# Autodesk Inventor assembly: Solar Array
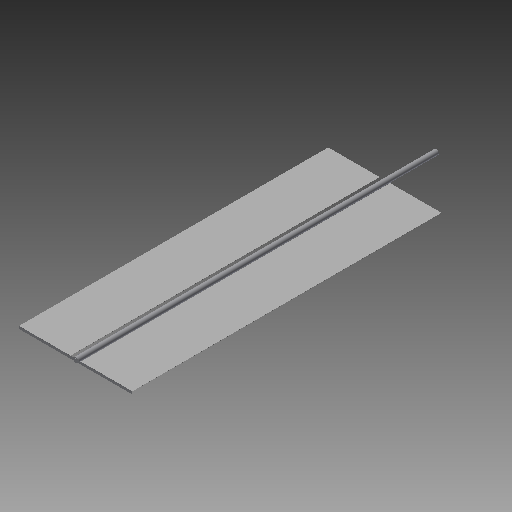
[picture p0: Inventor's stored thumbnail of the model, 512x512]
Saved by Autodesk Inventor 2017.2 (Build 212233000, 233)
## iProperties
Created: 2017-03-31
Part Number: Solar Array
Document SubType Name: Assembly
Designer: haden
Author: haden
## Documents named in this file (3)
- C:\Users\haden\Desktop\Asteroid-Mining-Project\CAD model\Solar Module\Solar Array.iam
- C:\Users\haden\Desktop\Asteroid-Mining-Project\CAD model\Solar Module\Long Rod.ipt
- C:\Users\haden\Desktop\Asteroid-Mining-Project\CAD model\Solar Module\Panel.ipt
## Components (3 placed, 2 different names)
1. Long Rod:1 — Flush:2, Flush:3, Mate:1, Flush:4
2. Panel:1 — Flush:1, Flush:2, Flush:5
3. Panel:2 — Flush:1, Flush:3, Mate:1, Flush:4, Flush:5
## Relationships (6: Flush 5, Mate 1)
- Flush:1: Panel:1 ↔ Panel:2
- Flush:2: Long Rod:1 ↔ Panel:1
- Flush:3: Long Rod:1 ↔ Panel:2
- Mate:1 (10 mm): Long Rod:1 ↔ Panel:2
- Flush:4: Long Rod:1 ↔ Panel:2
- Flush:5: Panel:1 ↔ Panel:2
